# Autodesk Inventor assembly: Skeleton V03
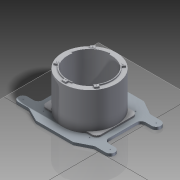
[picture p0: Inventor's stored thumbnail of the model, 180x180]
Saved by Autodesk Inventor 2015 (Build 190159000, 159)
## iProperties
Created: 2015-03-21
Part Number: Skeleton V03
Document SubType Name: Assembly
Designer: -
Author: -
## Documents named in this file (3)
- C:\Users\spichelh\Documents\GitHub\beta-hardware\Enclosure\SkeletonV03\Skeleton V03.iam
- C:\Users\spichelh\Documents\GitHub\beta-hardware\Enclosure\SkeletonV03\BetaSkeletonV01.ipt
- C:\Users\spichelh\Documents\GitHub\beta-hardware\Enclosure\SkeletonV03\F-mount to CMV12k-V05.ipt
## Components (2 placed, 2 different names)
1. BetaSkeletonV01:1 — Mate:7, Mate:8, Mate:9, Mate:10, Flush:3, Mate:11
2. F-mount to CMV12k-V05:1 — Mate:7, Mate:8, Mate:9, Mate:10, Flush:3
## Relationships (7: Mate 5, Flush 2)
- [Flush]: BetaSkeletonV01:1
- Mate:7: BetaSkeletonV01:1 ↔ F-mount to CMV12k-V05:1
- Mate:8: BetaSkeletonV01:1 ↔ F-mount to CMV12k-V05:1
- Mate:9: BetaSkeletonV01:1 ↔ F-mount to CMV12k-V05:1
- Mate:10: BetaSkeletonV01:1 ↔ F-mount to CMV12k-V05:1
- Flush:3: BetaSkeletonV01:1 ↔ F-mount to CMV12k-V05:1
- Mate:11: BetaSkeletonV01:1
